# Autodesk Inventor assembly: 組合檔
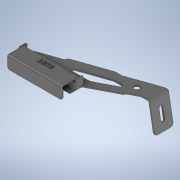
[picture p0: Inventor's stored thumbnail of the model, 180x180]
Saved by Autodesk Inventor 2022 (Build 260153000, 153)
## iProperties
Created: 2015-11-28
Part Number: 組合檔
Document SubType Name: Assembly
Designer: 設計製圖
Author: 設計製圖
## Documents named in this file (4)
- D:\資料庫\設計-3D Project\【May club 】\得利卡-車頂燈架\模型、圖面\成品版本\短-車頂燈架-組合(#01.05)\吊架-短(R)(#01.05)-完整.iam
- D:\資料庫\設計-3D Project\【May club 】\得利卡-車頂燈架\模型、圖面\成品版本\短-車頂燈架-組合(#01.05)\吊架-短(R)(#01.05) - 焊接組合.iam
- D:\資料庫\設計-3D Project\【May club 】\得利卡-車頂燈架\模型、圖面\成品版本\短-車頂燈架-組合(#01.05)\ㄇ槽(#01.05)- 焊接組合.iam
- C:\Users\p2013\OneDrive\桌面\補角片.ipt
## Components (3 placed, 3 different names)
1. 吊架-短(R)(#01.05) - 焊接組合:1 [sub-assembly] — 貼合:1, 貼合:2, 貼合:3, 齊平:2, 貼合:4
2. ㄇ槽(#01.05)- 焊接組合:1 [sub-assembly] — 貼合:1, 貼合:2
3. 補角片:1 — 貼合:3, 齊平:2, 貼合:4
## Relationships (6: Mate 4, Flush 2)
- 貼合:1 [Mate]: 吊架-短(R)(#01.05) - 焊接組合:1 ↔ ㄇ槽(#01.05)- 焊接組合:1
- 貼合:2 [Mate]: 吊架-短(R)(#01.05) - 焊接組合:1 ↔ ㄇ槽(#01.05)- 焊接組合:1
- 齊平:1 [Flush] (-120 mm)
- 貼合:3 [Mate]: 吊架-短(R)(#01.05) - 焊接組合:1 ↔ 補角片:1
- 齊平:2 [Flush]: 吊架-短(R)(#01.05) - 焊接組合:1 ↔ 補角片:1
- 貼合:4 [Mate]: 吊架-短(R)(#01.05) - 焊接組合:1 ↔ 補角片:1
